# Autodesk Inventor assembly: CA23[F]
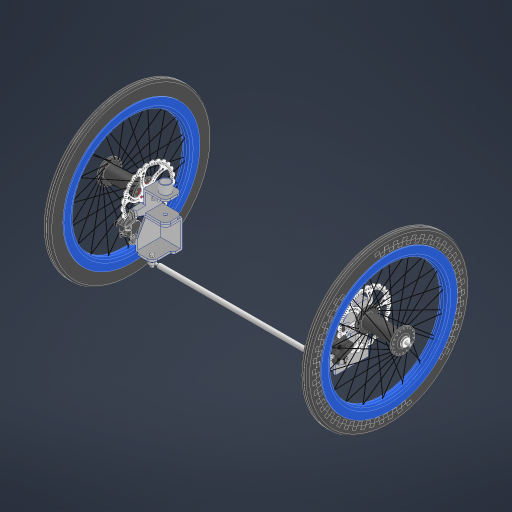
[picture p0: Inventor's stored thumbnail of the model, 512x512]
Saved by Autodesk Inventor 2024 (Build 280153000, 153)
## iProperties
Created: 2023-06-05
Part Number: CA23[F]
Document SubType Name: Assembly
Designer: juanj
Mass: 854.194 g
Surface Area: 1179.17 cm^2
Volume: 316.368 cm^3
Density: 2.7 g/cm^3
Author: juanj
## Documents named in this file (11)
- C:\Users\juanj\Documents\Documentos\Unisabana\Shell\C23 DESING\A23[F]\PFA23[F]\CA23[F].iam
- C:\Users\juanj\Documents\Documentos\Unisabana\Shell\C23 DESING\A23[F]\PFA23[F]\C23[i3][L][2].ipt
- C:\Users\juanj\Documents\Documentos\Unisabana\Shell\C23 DESING\A23[F]\PFA23[F]\C23[i3][R][1].ipt
- C:\Users\juanj\Documents\Documentos\Unisabana\Shell\C23 DESING\A23[F]\PFA23[F]\DC23[L][F][1].ipt
- C:\Users\juanj\Documents\Documentos\Unisabana\Shell\C23 DESING\A23[F]\PFA23[F]\DC23[R][F][1].ipt
- C:\Users\juanj\Documents\Documentos\Unisabana\Shell\C23 DESING\A23[F]\PFA23[F]\B23[F]_MIR2.ipt
- C:\Users\juanj\Documents\Documentos\Unisabana\Shell\C23 DESING\A23[F]\PFA23[F]\B23[F1].ipt
- C:\Users\juanj\Documents\Documentos\Unisabana\Shell\C23 DESING\A23[F]\PFA23[F]\HB[F].ipt
- C:\Users\juanj\Documents\Documentos\Unisabana\Shell\C23 DESING\A23[F]\PFA23[F]\D23[F].iam
- C:\Users\juanj\Documents\Documentos\Unisabana\Shell\C23 DESING\A23[F]\PFA23[F]\BU23[F].ipt
- C:\Users\juanj\Documents\Documentos\Unisabana\Shell\C23 DESING\A23[F]\PFA23[F]\W23[F].ipt
## Components (13 placed, 10 different names)
1. C23[i3][L][2]:1 — Insert:5, Angle:7, Insert:11
2. C23[i3][R][1]:1 — Insert:6, Angle:6, Insert:10
3. DC23[L][F][1]:1 — Insert:5, Angle:7, Insert:7, Angle:8, Mate:1, Angle:10, Mate:2
4. DC23[R][F][1]:1 — Insert:6, Angle:6, Insert:8, Angle:9, Insert:9, Angle:10
5. B23[F]_MIR2:1 — Insert:3, Angle:4, Insert:8, Angle:9
6. B23[F1]:1 — Insert:4, Angle:5, Insert:7, Angle:8
7. HB[F]:1 — Insert:4, Angle:5
8. HB[F]:2 — Insert:3, Angle:4
9. D23[F]:1 [sub-assembly] — Insert:9, Mate:1, Mate:2
10. BU23[F]:1 — Insert:11, Insert:12
11. W23[F]:1 — Insert:13
12. W23[F]:2 — Insert:12
13. BU23[F]:2 — Insert:10, Insert:13
## Relationships (20: Insert 11, Angle 7, Mate 2)
- Insert:3: B23[F]_MIR2:1 ↔ HB[F]:2
- Insert:4: B23[F1]:1 ↔ HB[F]:1
- Angle:4 (0 deg): B23[F]_MIR2:1 ↔ HB[F]:2
- Angle:5 (0 deg): B23[F1]:1 ↔ HB[F]:1
- Insert:5: C23[i3][L][2]:1 ↔ DC23[L][F][1]:1
- Insert:6: C23[i3][R][1]:1 ↔ DC23[R][F][1]:1
- Angle:6 (0 deg): C23[i3][R][1]:1 ↔ DC23[R][F][1]:1
- Angle:7 (0 deg): C23[i3][L][2]:1 ↔ DC23[L][F][1]:1
- Insert:7: DC23[L][F][1]:1 ↔ B23[F1]:1
- Angle:8 (0 deg): DC23[L][F][1]:1 ↔ B23[F1]:1
- Insert:8: DC23[R][F][1]:1 ↔ B23[F]_MIR2:1
- Angle:9 (0 deg): DC23[R][F][1]:1 ↔ B23[F]_MIR2:1
- Insert:9: DC23[R][F][1]:1 ↔ D23[F]:1
- Mate:1: DC23[L][F][1]:1 ↔ D23[F]:1
- Angle:10 (0 deg): DC23[L][F][1]:1 ↔ DC23[R][F][1]:1
- Mate:2: DC23[L][F][1]:1 ↔ D23[F]:1
- Insert:10: C23[i3][R][1]:1 ↔ BU23[F]:2
- Insert:11: C23[i3][L][2]:1 ↔ BU23[F]:1
- Insert:12: BU23[F]:1 ↔ W23[F]:2
- Insert:13: W23[F]:1 ↔ BU23[F]:2
